# Autodesk Inventor assembly: Крепления и направляющие
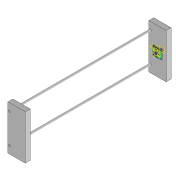
[picture p0: Inventor's stored thumbnail of the model, 180x180]
Saved by Autodesk Inventor 2022 (Build 260153000, 153)
## iProperties
Created: 2023-02-20
Part Number: Крепления и направляющие
Document SubType Name: Assembly
Designer: Глеб
Author: Глеб
## Documents named in this file (4)
- C:\Users\Глеб\Documents\Inventor\Файлы Inventor\Крепления и направляющие.iam
- C:\Users\Глеб\Documents\Inventor\Файлы Inventor\Крепление для опор.ipt
- C:\Users\Глеб\Documents\Inventor\Файлы Inventor\Опора подъемника.ipt
- C:\Users\Глеб\Documents\Inventor\Файлы Inventor\Ov5647 камера.ipt
## Components (5 placed, 3 different names)
1. Ov5647 камера:1 — Совмещение:8
2. Крепление для опор:1 — Совмещение:1, Совмещение:2, Совмещение:5, Совмещение:6, Совмещение:8
3. Опора подъемника:1 — Совмещение:1, Совмещение:3, Совмещение:6
4. Опора подъемника:2 — Совмещение:2, Совмещение:4, Совмещение:5, Совмещение:7, Заподлицо:1
5. Крепление для опор:2 — Совмещение:3, Совмещение:4, Совмещение:7, Заподлицо:1
## Relationships (9: Mate 8, Flush 1)
- Совмещение:1 [Mate]: Крепление для опор:1 ↔ Опора подъемника:1
- Совмещение:2 [Mate]: Крепление для опор:1 ↔ Опора подъемника:2
- Совмещение:3 [Mate]: Опора подъемника:1 ↔ Крепление для опор:2
- Совмещение:4 [Mate]: Опора подъемника:2 ↔ Крепление для опор:2
- Совмещение:5 [Mate]: Крепление для опор:1 ↔ Опора подъемника:2
- Совмещение:6 [Mate]: Крепление для опор:1 ↔ Опора подъемника:1
- Совмещение:7 [Mate]: Опора подъемника:2 ↔ Крепление для опор:2
- Заподлицо:1 [Flush]: Опора подъемника:2 ↔ Крепление для опор:2
- Совмещение:8 [Mate]: Ov5647 камера:1 ↔ Крепление для опор:1
